# Autodesk Inventor assembly: Gripper_Link
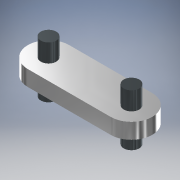
[picture p0: Inventor's stored thumbnail of the model, 180x180]
Saved by Autodesk Inventor 2021.3 (Build 253353000, 353)
## iProperties
Created: 2021-04-16
Part Number: Gripper_Link
Document SubType Name: Assembly
Designer: domin
Author: domin
## Documents named in this file (3)
- E:\Transfer\Sync\Hivemind\1-MCI-Unterlagen\Master\Semester 2\Projekt 1\Hausberger\Workfolder_Dommy\Gripper\Gripper_Link.iam
- E:\Transfer\Sync\Hivemind\1-MCI-Unterlagen\Master\Semester 2\Projekt 1\Hausberger\Workfolder_Dommy\Gripper\Gripper_Link.ipt
- E:\Transfer\Sync\Hivemind\1-MCI-Unterlagen\Master\Semester 2\Projekt 1\Hausberger\Workfolder_Dommy\Gripper\Bolt_3_10.ipt
## Components (3 placed, 2 different names)
1. Gripper_Link:1 — Mate:1, Mate:2, Mate:3, Mate:4, Mate:5, Flush:1, Flush:2
2. Bolt_3_10:1 — Mate:4, Flush:1
3. Bolt_3_10:2 — Mate:5, Flush:2
## Relationships (7: Mate 5, Flush 2)
- Mate:1: Gripper_Link:1
- Mate:2: Gripper_Link:1
- Mate:3: Gripper_Link:1
- Mate:4: Gripper_Link:1 ↔ Bolt_3_10:1
- Mate:5: Gripper_Link:1 ↔ Bolt_3_10:2
- Flush:1 (-3.5 mm): Gripper_Link:1 ↔ Bolt_3_10:1
- Flush:2 (-3.5 mm): Gripper_Link:1 ↔ Bolt_3_10:2
